# Autodesk Inventor assembly: Head
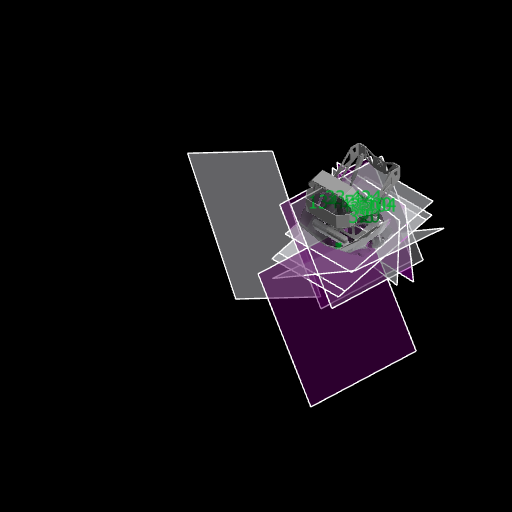
[picture p0: Inventor's stored thumbnail of the model, 512x512]
Saved by Autodesk Inventor 2025.2 (Build 292293000, 293)
## iProperties
Created: 2024-12-17
Part Number: Head
Document SubType Name: Assembly
Designer: valer
Author: valer
## Documents named in this file (47)
- C:\Users\valer\Desktop\str1ker\cad\Head.iam
- C:\Users\valer\Desktop\str1ker\cad\Head.ipt
- C:\Users\valer\Desktop\str1ker\cad\HeadMount.ipt
- C:\Users\valer\Desktop\str1ker\cad\external\DepthSensor\PrimeSenseCarmine1.09.ipt
- C:\Users\valer\Desktop\str1ker\cad\external\HingedThreadedStandoffPart1.ipt
- C:\Users\valer\Desktop\str1ker\cad\external\HingedThreadedStandoffPart2.ipt
- C:\Users\valer\Desktop\str1ker\cad\external\ShaftD6Female-632Female.ipt
- C:\Users\valer\Desktop\str1ker\cad\external\ShaftD6-2101-0006-0160.ipt
- C:\Users\valer\Desktop\str1ker\cad\TongueMount.ipt
- C:\Users\valer\Desktop\str1ker\cad\external\SetScrewLiteHub-1308-0016-0006.ipt
- C:\Users\valer\Desktop\str1ker\cad\external\ShaftD6-Short-2101-0006-0020.ipt
- C:\Users\valer\Desktop\str1ker\cad\external\UJoint6D\UJoint6D-Body-4003-1006-1006.ipt
- C:\Users\valer\Desktop\str1ker\cad\external\UJoint6D\UJoint6D-Screw.ipt
- C:\Users\valer\Desktop\str1ker\cad\external\UJoint6D\UJoint6D-CenterDrive-4003-1006-1006.ipt
- C:\Users\valer\Desktop\str1ker\cad\external\ShaftD6-2100-0006-0200.ipt
- C:\Users\valer\Desktop\str1ker\cad\external\ShaftD6-2101-0006-0140.ipt
- C:\Users\valer\Desktop\str1ker\cad\external\LinearBearing-1612-0612-0035.ipt
- C:\Users\valer\Desktop\str1ker\cad\external\ClampingHub1301-0016-0012.ipt
- C:\Users\valer\Desktop\str1ker\cad\external\ShaftClamp6-6058N14.ipt
- C:\Users\valer\Desktop\str1ker\cad\external\TongueSpeaker.ipt
- C:\Users\valer\Desktop\str1ker\cad\TongueSideLid.ipt
- C:\Users\valer\Desktop\str1ker\cad\TongueSideLidMirror.ipt
- C:\Users\valer\Desktop\str1ker\cad\NoseMount.ipt
- C:\Users\valer\Desktop\str1ker\cad\JawMount.ipt
- C:\Users\valer\Desktop\str1ker\cad\external\93655A703_Male-Female Threaded Hex Standoff.ipt
- C:\Users\valer\Desktop\str1ker\cad\CameraMount.ipt
- C:\Users\valer\Desktop\str1ker\cad\external\ServoHorn-1900-0024-0104.ipt
- C:\Users\valer\Desktop\str1ker\cad\external\ServoCity-2000-0025-0002.ipt
- C:\Users\valer\Desktop\str1ker\cad\external\Beam4-1102-0004-0032.ipt
- C:\Users\valer\Desktop\str1ker\cad\Visor.ipt
- C:\Users\valer\Desktop\str1ker\cad\external\NeckActuator\LA-T8-1215-50 105-64 Body.ipt
- C:\Users\valer\Desktop\str1ker\cad\external\NeckActuator\LA-T8-1215-50 105-64 Shaft.ipt
- C:\Users\valer\Desktop\str1ker\cad\external\NeckActuator\LA-T8-Bracket.ipt
- C:\Users\valer\Desktop\str1ker\cad\NeckBase.ipt
- C:\Users\valer\Desktop\str1ker\cad\NeckBracket.ipt
- C:\Users\valer\Desktop\str1ker\cad\NeckBracketMirror.ipt
- C:\Users\valer\Desktop\str1ker\cad\NeckCover.ipt
- C:\Users\valer\Desktop\str1ker\cad\NeckPotentiometerBracket.ipt
- C:\Users\valer\Desktop\str1ker\cad\external\PololuHub1994.ipt
- C:\Users\valer\Desktop\str1ker\cad\external\rh24pce.iam
- C:\Users\valer\Desktop\str1ker\cad\NeckMiddleBracket.ipt
- C:\Users\valer\Desktop\str1ker\cad\external\Hub8mm.ipt
- C:\Users\valer\Desktop\str1ker\cad\external\am-4180 Lamprey Absolute Encoder Magnet Ring.ipt
- C:\Users\valer\Desktop\str1ker\cad\NeckRingAlign.ipt
- C:\Users\valer\Desktop\str1ker\cad\external\Max9744_20W_ClassD_Amplifier.ipt
- C:\Users\valer\Desktop\str1ker\cad\external\StepperDriver\HiLetgoTB6600HG.ipt
- C:\Users\valer\Desktop\str1ker\cad\external\ArmDriver\IBTMini.ipt
## Components (94 placed, 46 different names)
1. Head:1 — Flush:1, Flush:2, Mate:1, Flush:3, Mate:4, Mate:5, Mate:6, Mate:7, Mate:8, Mate:9, Mate:10, Mate:11, Mate:12, Mate:13, Mate:14, Mate:15, Mate:16, Mate:17, Mate:18, Mate:19, Mate:20, Mate:59, Angle:13, Mate:89, Mate:90, Flush:13, Mate:119, Mate:121, Flush:15, Flush:16, Flush:17, Flush:18, Flush:19, Mate:124, Mate:125, Mate:126, Mate:127, Mate:128, Mate:129, Flush:20, Mate:131, Mate:132, Mate:133, Flush:157, Flush:166, Mate:230
2. HeadMount:1 — Flush:4, Flush:5, Angle:18, Mate:89, Mate:90, Angle:20, Angle:22, Angle:26, Angle:28, Angle:32, Mate:102, Mate:105, Mate:107, Mate:109, Mate:111, Mate:113, Mate:115, Mate:134, Mate:135, Mate:136, Mate:137, Angle:35, Mate:167, Flush:158, Mate:178, Mate:189, Mate:192, Mate:193, Mate:194, Mate:195, Angle:37, Angle:39, Angle:40, Mate:215, Angle:42, Mate:216
3. PrimeSenseCarmine1.09:1 — Flush:6, Flush:23, Mate:138, Mate:198
4. HingedThreadedStandoffPart1:1 — Mate:4, Mate:5, Mate:25, Mate:26
5. HingedThreadedStandoffPart1:2 — Mate:6, Mate:7, Mate:36, Mate:39
6. HingedThreadedStandoffPart1:3 — Mate:8, Mate:9, Mate:37, Mate:38
7. HingedThreadedStandoffPart1:4 — Mate:10, Mate:11, Mate:23, Mate:24
8. HingedThreadedStandoffPart1:5 — Mate:12, Mate:13, Mate:27, Mate:28
9. HingedThreadedStandoffPart1:6 — Mate:16, Mate:17, Mate:29, Mate:40
10. HingedThreadedStandoffPart1:7 — Mate:14, Mate:15, Mate:30, Mate:31
11. HingedThreadedStandoffPart1:8 — Mate:18, Mate:19, Mate:32, Mate:34
12. HingedThreadedStandoffPart1:9 — Mate:20, Mate:33, Mate:35, Mate:59
13. HingedThreadedStandoffPart2:4 — Mate:23, Mate:24, Flush:7, Flush:8
14. HingedThreadedStandoffPart2:5 — Mate:25, Mate:26, Flush:8, Mate:68
15. HingedThreadedStandoffPart2:6 — Mate:27, Mate:28, Flush:7, Flush:10, Mate:69
16. HingedThreadedStandoffPart2:7 — Mate:29, Mate:40, Mate:45, Mate:47
17. HingedThreadedStandoffPart2:8 — Mate:30, Mate:31, Mate:46, Mate:48
18. HingedThreadedStandoffPart2:9 — Mate:32, Mate:34, Mate:49, Mate:52
19. HingedThreadedStandoffPart2:10 — Mate:33, Mate:35, Mate:50, Mate:51
20. HingedThreadedStandoffPart2:11 — Mate:36, Mate:39, Mate:41, Mate:42
21. HingedThreadedStandoffPart2:12 — Mate:37, Mate:38, Mate:43, Mate:44
22. ShaftD6-2100-0006-0200:1 — Mate:87, Angle:17, Mate:88, Angle:18, Mate:108
23. ShaftD6Female-632Female:1 — Mate:41, Mate:42, Mate:87, Angle:17, Mate:88
24. ShaftD6Female-632Female:2 — Mate:43, Mate:44, Mate:91, Mate:92
25. ShaftD6Female-632Female:3 — Mate:45, Mate:47, Mate:95, Mate:96, Angle:23
26. ShaftD6Female-632Female:4 — Mate:46, Mate:48, Mate:93, Mate:94, Angle:21
27. ShaftD6Female-632Female:5 — Mate:49, Mate:52, Mate:99, Mate:100, Angle:30
28. ShaftD6Female-632Female:6 — Mate:50, Mate:51, Mate:97, Mate:98, Angle:27
29. TongueMount:1 — Flush:11, Mate:66, Mate:67, Angle:11, Mate:68, Mate:69, Mate:71
30. SetScrewLiteHub-1308-0016-0006:1 — Mate:66, Mate:67, Angle:11, Mate:70, Mate:73
31. ShaftD6-Short-2101-0006-0020:1 — Mate:70, Mate:71, Mate:72, Angle:12
32. UJoint6D-Body-4003-1006-1006:1 — Mate:72, Mate:73, Angle:12, Mate:74, Mate:75, Mate:76, Mate:77, Mate:78, Mate:79
33. UJoint6D-Screw:1 — Mate:82, Mate:83
34. UJoint6D-CenterDrive-4003-1006-1006:1 — Mate:74, Mate:75, Mate:80, Mate:81
35. UJoint6D-Screw:2 — Mate:76, Mate:77
36. UJoint6D-Screw:3 — Mate:78, Mate:79
37. UJoint6D-Body-4003-1006-1006:2 — Mate:80, Mate:81, Angle:13, Mate:82, Mate:83, Mate:84, Mate:85, Mate:86, Angle:14, Flush:12
38. UJoint6D-Screw:4 — Mate:84, Mate:85
39. ShaftD6-2101-0006-0160:7 — Mate:86, Angle:14, Flush:12, Mate:101, Mate:166, Mate:168
40. ShaftD6-2100-0006-0200:2 — Mate:91, Mate:92, Angle:19, Angle:20, Mate:110
41. ShaftD6-2101-0006-0140:1 — Mate:93, Mate:94, Angle:21, Angle:22, Angle:24, Mate:104
42. ShaftD6-2101-0006-0140:2 — Mate:95, Mate:96, Angle:23, Angle:25, Angle:26, Mate:106
43. ShaftD6-2101-0006-0140:3 — Mate:97, Mate:98, Angle:27, Angle:28, Angle:29, Mate:112
44. ShaftD6-2101-0006-0140:4 — Mate:99, Mate:100, Angle:30, Angle:31, Angle:32, Mate:114
45. LinearBearing-1612-0612-0035:1 — Mate:101, Mate:103, Flush:160
46. ClampingHub1301-0016-0012:1 — Mate:102, Mate:103, Flush:160, Mate:197, Angle:37
47. ShaftClamp6-6058N14:1 — Mate:106, Mate:107
48. ShaftClamp6-6058N14:2 — Mate:104, Mate:105
49. ShaftClamp6-6058N14:3 — Mate:108, Mate:109
50. ShaftClamp6-6058N14:4 — Mate:110, Mate:111
51. ShaftClamp6-6058N14:5 — Mate:114, Mate:115
52. ShaftClamp6-6058N14:6 — Mate:112, Mate:113
53. TongueSpeaker:1 — Mate:119, Mate:122, Mate:123
54. TongueSpeaker:2 — Mate:121, Mate:130
55. TongueSideLid:1 — Mate:124, Mate:125, Mate:126
56. TongueSideLidMirror:1 — Mate:127, Mate:128, Mate:129, Mate:130
57. NoseMount:1 — Flush:21, Mate:131, Mate:132, Mate:133
58. JawMount:1 — Flush:22
59. 93655A703_Male-Female Threaded Hex Standoff:1 — Mate:134, Mate:136, Mate:141, Mate:143
60. 93655A703_Male-Female Threaded Hex Standoff:2 — Mate:135, Mate:137, Mate:142
61. CameraMount:1 — Flush:24, Mate:138, Mate:141, Mate:142, Mate:143, Mate:198
62. ServoHorn-1900-0024-0104:1 — Mate:164, Mate:165, Mate:169, Mate:170
63. ServoCity-2000-0025-0002:1 — Mate:164, Mate:165, Angle:35, Flush:153, Mate:167
64. ShaftClamp6-6058N14:7 — Mate:166, Mate:197
65. ShaftClamp6-6058N14:8 — Mate:168, Mate:171
66. Beam4-1102-0004-0032:1 — Mate:169, Mate:170, Mate:171
67. Visor:1 — Flush:157, Flush:158, Mate:178
68. LA-T8-1215-50 105-64 Body:1 — Mate:172, Mate:175, Mate:179, Mate:180
69. LA-T8-1215-50 105-64 Shaft:1 — Mate:172, Mate:175, Mate:181, Mate:182
70. LA-T8-Bracket:1 — Mate:181, Mate:182, Mate:192, Mate:194, Mate:195, Angle:40
71. LA-T8-Bracket:2 — Mate:179, Mate:180, Mate:206, Mate:237, Angle:47
72. LA-T8-1215-50 105-64 Body:2
73. LA-T8-1215-50 105-64 Shaft:2
74. LA-T8-Bracket:3 — Mate:189, Mate:193, Angle:39
75. LA-T8-Bracket:4 — Mate:238, Angle:46, Mate:249
76. NeckBracket:1 — Mate:206, Mate:237, Mate:239, Mate:240, Mate:241, Mate:244, Angle:47
77. NeckCover:1 — Flush:166
78. NeckCover:2 — Mate:244, Mate:250, Mate:251
79. NeckPotentiometerBracket:1 — Mate:215, Angle:42, Angle:43, Flush:167, Mate:217, Mate:218, Mate:219, Mate:227, Mate:268
80. NeckPotentiometerBracket:2 — Angle:43, Mate:216, Flush:167, Mate:220, Mate:221, Mate:222, Mate:228, Mate:229
81. PololuHub1994:1 — Mate:217, Mate:218, Mate:219
82. PololuHub1994:2 — Mate:220, Mate:221, Mate:222
83. NeckPotentiometerBracket:3 — Mate:227, Flush:168, Mate:268, Mate:269, Mate:270
84. NeckPotentiometerBracket:4 — Mate:228, Mate:229, Flush:168, Mate:266
85. NeckMiddleBracket:1 — Mate:230, Mate:257, Flush:172, Flush:173, Mate:266, Mate:271, Mate:272, Angle:50, Angle:51, Mate:273, Flush:174, Flush:175, Flush:176
86. Hub8mm:1 — Mate:254, Mate:258, Mate:259, Mate:261, Mate:263, Mate:264
87. NeckBase:1 — Mate:238, Mate:239, Mate:240, Mate:241, Mate:246, Mate:247, Mate:248, Mate:254, Mate:255, Mate:258, Mate:259, Mate:262
88. NeckBracketMirror:1 — Mate:246, Mate:247, Mate:248, Angle:46, Mate:249, Mate:250, Mate:251, Mate:257, Flush:172, Flush:173, Mate:275
89. am-4180 Lamprey Absolute Encoder Magnet Ring:1 — Mate:255, Mate:263
90. NeckRingAlign:1 — Mate:261, Mate:262, Mate:264
91. rh24pce:1 [sub-assembly] — Mate:269, Mate:270
92. Max9744_20W_ClassD_Amplifier:1 — Mate:272, Angle:51, Mate:275, Flush:176
93. HiLetgoTB6600HG:1 — Mate:271, Angle:50, Mate:274, Flush:175
94. IBTMini:1 — Mate:273, Mate:274, Flush:174
## Relationships (258: Mate 192, Flush 34, Angle 30, Symmetry 2)
- Flush:1: Head:1
- Flush:2: Head:1
- Mate:1: Head:1
- Flush:3: Head:1
- Flush:4: HeadMount:1
- Flush:5: HeadMount:1
- Flush:6: PrimeSenseCarmine1.09:1
- Mate:4: Head:1 ↔ HingedThreadedStandoffPart1:1
- Mate:5: Head:1 ↔ HingedThreadedStandoffPart1:1
- Mate:6: Head:1 ↔ HingedThreadedStandoffPart1:2
- Mate:7: Head:1 ↔ HingedThreadedStandoffPart1:2
- Mate:8: Head:1 ↔ HingedThreadedStandoffPart1:3
- Mate:9: Head:1 ↔ HingedThreadedStandoffPart1:3
- Mate:10: Head:1 ↔ HingedThreadedStandoffPart1:4
- Mate:11: Head:1 ↔ HingedThreadedStandoffPart1:4
- Mate:12: Head:1 ↔ HingedThreadedStandoffPart1:5
- Mate:13: Head:1 ↔ HingedThreadedStandoffPart1:5
- Mate:14: Head:1 ↔ HingedThreadedStandoffPart1:7
- Mate:15: Head:1 ↔ HingedThreadedStandoffPart1:7
- Mate:16: Head:1 ↔ HingedThreadedStandoffPart1:6
- Mate:17: Head:1 ↔ HingedThreadedStandoffPart1:6
- Mate:18: Head:1 ↔ HingedThreadedStandoffPart1:8
- Mate:19: Head:1 ↔ HingedThreadedStandoffPart1:8
- Mate:20: Head:1 ↔ HingedThreadedStandoffPart1:9
- Mate:23: HingedThreadedStandoffPart1:4 ↔ HingedThreadedStandoffPart2:4
- Mate:24: HingedThreadedStandoffPart1:4 ↔ HingedThreadedStandoffPart2:4
- Mate:25: HingedThreadedStandoffPart1:1 ↔ HingedThreadedStandoffPart2:5
- Mate:26: HingedThreadedStandoffPart1:1 ↔ HingedThreadedStandoffPart2:5
- Mate:27: HingedThreadedStandoffPart1:5 ↔ HingedThreadedStandoffPart2:6
- Mate:28: HingedThreadedStandoffPart1:5 ↔ HingedThreadedStandoffPart2:6
- Mate:29: HingedThreadedStandoffPart1:6 ↔ HingedThreadedStandoffPart2:7
- Mate:30: HingedThreadedStandoffPart1:7 ↔ HingedThreadedStandoffPart2:8
- Mate:31: HingedThreadedStandoffPart1:7 ↔ HingedThreadedStandoffPart2:8
- Mate:32: HingedThreadedStandoffPart1:8 ↔ HingedThreadedStandoffPart2:9
- Mate:33: HingedThreadedStandoffPart1:9 ↔ HingedThreadedStandoffPart2:10
- Mate:34: HingedThreadedStandoffPart1:8 ↔ HingedThreadedStandoffPart2:9
- Mate:35: HingedThreadedStandoffPart1:9 ↔ HingedThreadedStandoffPart2:10
- Mate:36: HingedThreadedStandoffPart1:2 ↔ HingedThreadedStandoffPart2:11
- Mate:37: HingedThreadedStandoffPart1:3 ↔ HingedThreadedStandoffPart2:12
- Mate:38: HingedThreadedStandoffPart1:3 ↔ HingedThreadedStandoffPart2:12
- Mate:39: HingedThreadedStandoffPart1:2 ↔ HingedThreadedStandoffPart2:11
- Mate:40: HingedThreadedStandoffPart1:6 ↔ HingedThreadedStandoffPart2:7
- Flush:7: HingedThreadedStandoffPart2:4 ↔ HingedThreadedStandoffPart2:6
- Flush:8: HingedThreadedStandoffPart2:4 ↔ HingedThreadedStandoffPart2:5
- Mate:41: HingedThreadedStandoffPart2:11 ↔ ShaftD6Female-632Female:1
- Mate:42: HingedThreadedStandoffPart2:11 ↔ ShaftD6Female-632Female:1
- Mate:43: HingedThreadedStandoffPart2:12 ↔ ShaftD6Female-632Female:2
- Mate:44: HingedThreadedStandoffPart2:12 ↔ ShaftD6Female-632Female:2
- Mate:45: HingedThreadedStandoffPart2:7 ↔ ShaftD6Female-632Female:3
- Mate:46: HingedThreadedStandoffPart2:8 ↔ ShaftD6Female-632Female:4
- Mate:47: HingedThreadedStandoffPart2:7 ↔ ShaftD6Female-632Female:3
- Mate:48: HingedThreadedStandoffPart2:8 ↔ ShaftD6Female-632Female:4
- Mate:49: HingedThreadedStandoffPart2:9 ↔ ShaftD6Female-632Female:5
- Mate:50: HingedThreadedStandoffPart2:10 ↔ ShaftD6Female-632Female:6
- Mate:51: HingedThreadedStandoffPart2:10 ↔ ShaftD6Female-632Female:6
- Mate:52: HingedThreadedStandoffPart2:9 ↔ ShaftD6Female-632Female:5
- Mate:59: Head:1 ↔ HingedThreadedStandoffPart1:9
- Flush:10: HingedThreadedStandoffPart2:6
- Flush:11: TongueMount:1
- Mate:66: TongueMount:1 ↔ SetScrewLiteHub-1308-0016-0006:1
- Mate:67: TongueMount:1 ↔ SetScrewLiteHub-1308-0016-0006:1
- Angle:11 (0 deg): TongueMount:1 ↔ SetScrewLiteHub-1308-0016-0006:1
- Mate:68: HingedThreadedStandoffPart2:5 ↔ TongueMount:1
- Mate:69: HingedThreadedStandoffPart2:6 ↔ TongueMount:1
- Mate:70: SetScrewLiteHub-1308-0016-0006:1 ↔ ShaftD6-Short-2101-0006-0020:1
- Mate:71: TongueMount:1 ↔ ShaftD6-Short-2101-0006-0020:1
- Mate:72: ShaftD6-Short-2101-0006-0020:1 ↔ UJoint6D-Body-4003-1006-1006:1
- Mate:73: SetScrewLiteHub-1308-0016-0006:1 ↔ UJoint6D-Body-4003-1006-1006:1
- Angle:12 (0 deg): ShaftD6-Short-2101-0006-0020:1 ↔ UJoint6D-Body-4003-1006-1006:1
- Mate:74: UJoint6D-Body-4003-1006-1006:1 ↔ UJoint6D-CenterDrive-4003-1006-1006:1
- Mate:75: UJoint6D-Body-4003-1006-1006:1 ↔ UJoint6D-CenterDrive-4003-1006-1006:1
- Mate:76: UJoint6D-Body-4003-1006-1006:1 ↔ UJoint6D-Screw:2
- Mate:77: UJoint6D-Body-4003-1006-1006:1 ↔ UJoint6D-Screw:2
- Mate:78: UJoint6D-Body-4003-1006-1006:1 ↔ UJoint6D-Screw:3
- Mate:79: UJoint6D-Body-4003-1006-1006:1 ↔ UJoint6D-Screw:3
- Mate:80: UJoint6D-CenterDrive-4003-1006-1006:1 ↔ UJoint6D-Body-4003-1006-1006:2
- Mate:81: UJoint6D-CenterDrive-4003-1006-1006:1 ↔ UJoint6D-Body-4003-1006-1006:2
- Angle:13 (0 deg): Head:1 ↔ UJoint6D-Body-4003-1006-1006:2
- Mate:82: UJoint6D-Screw:1 ↔ UJoint6D-Body-4003-1006-1006:2
- Mate:83: UJoint6D-Screw:1 ↔ UJoint6D-Body-4003-1006-1006:2
- Mate:84: UJoint6D-Body-4003-1006-1006:2 ↔ UJoint6D-Screw:4
- Mate:85: UJoint6D-Body-4003-1006-1006:2 ↔ UJoint6D-Screw:4
- Mate:86: UJoint6D-Body-4003-1006-1006:2 ↔ ShaftD6-2101-0006-0160:7
- Angle:14 (180 deg): UJoint6D-Body-4003-1006-1006:2 ↔ ShaftD6-2101-0006-0160:7
- Flush:12: UJoint6D-Body-4003-1006-1006:2 ↔ ShaftD6-2101-0006-0160:7
- Mate:87: ShaftD6-2100-0006-0200:1 ↔ ShaftD6Female-632Female:1
- Angle:17 (0 deg): ShaftD6-2100-0006-0200:1 ↔ ShaftD6Female-632Female:1
- Mate:88: ShaftD6-2100-0006-0200:1 ↔ ShaftD6Female-632Female:1
- Angle:18 (0 deg): HeadMount:1 ↔ ShaftD6-2100-0006-0200:1
- Mate:89: Head:1 ↔ HeadMount:1
- Mate:90: Head:1 ↔ HeadMount:1
- Mate:91: ShaftD6Female-632Female:2 ↔ ShaftD6-2100-0006-0200:2
- Mate:92: ShaftD6Female-632Female:2 ↔ ShaftD6-2100-0006-0200:2
- Angle:19 (0 deg): ShaftD6-2100-0006-0200:2
- Angle:20 (0 deg): HeadMount:1 ↔ ShaftD6-2100-0006-0200:2
- Mate:93: ShaftD6Female-632Female:4 ↔ ShaftD6-2101-0006-0140:1
- Mate:94: ShaftD6Female-632Female:4 ↔ ShaftD6-2101-0006-0140:1
- Angle:21 (0 deg): ShaftD6Female-632Female:4 ↔ ShaftD6-2101-0006-0140:1
- Angle:22 (0 deg): HeadMount:1 ↔ ShaftD6-2101-0006-0140:1
- Mate:95: ShaftD6Female-632Female:3 ↔ ShaftD6-2101-0006-0140:2
- Mate:96: ShaftD6Female-632Female:3 ↔ ShaftD6-2101-0006-0140:2
- Angle:23 (0 deg): ShaftD6Female-632Female:3 ↔ ShaftD6-2101-0006-0140:2
- Angle:24 (180 deg): ShaftD6-2101-0006-0140:1
- Angle:25 (180 deg): ShaftD6-2101-0006-0140:2
- Angle:26 (0 deg): HeadMount:1 ↔ ShaftD6-2101-0006-0140:2
- Mate:97: ShaftD6Female-632Female:6 ↔ ShaftD6-2101-0006-0140:3
- Mate:98: ShaftD6Female-632Female:6 ↔ ShaftD6-2101-0006-0140:3
- Angle:27 (0 deg): ShaftD6Female-632Female:6 ↔ ShaftD6-2101-0006-0140:3
- Angle:28 (0 deg): HeadMount:1 ↔ ShaftD6-2101-0006-0140:3
- Angle:29 (0 deg): ShaftD6-2101-0006-0140:3
- Mate:99: ShaftD6Female-632Female:5 ↔ ShaftD6-2101-0006-0140:4
- Mate:100: ShaftD6Female-632Female:5 ↔ ShaftD6-2101-0006-0140:4
- Angle:30 (0 deg): ShaftD6Female-632Female:5 ↔ ShaftD6-2101-0006-0140:4
- Angle:31 (0 deg): ShaftD6-2101-0006-0140:4
- Angle:32 (0 deg): HeadMount:1 ↔ ShaftD6-2101-0006-0140:4
- Mate:101: ShaftD6-2101-0006-0160:7 ↔ LinearBearing-1612-0612-0035:1
- Mate:102: HeadMount:1 ↔ ClampingHub1301-0016-0012:1
- Mate:103: LinearBearing-1612-0612-0035:1 ↔ ClampingHub1301-0016-0012:1
- Mate:104: ShaftD6-2101-0006-0140:1 ↔ ShaftClamp6-6058N14:2
- Mate:105: HeadMount:1 ↔ ShaftClamp6-6058N14:2
- Mate:106: ShaftD6-2101-0006-0140:2 ↔ ShaftClamp6-6058N14:1
- Mate:107: HeadMount:1 ↔ ShaftClamp6-6058N14:1
- Mate:108: ShaftD6-2100-0006-0200:1 ↔ ShaftClamp6-6058N14:3
- Mate:109: HeadMount:1 ↔ ShaftClamp6-6058N14:3
- Mate:110: ShaftD6-2100-0006-0200:2 ↔ ShaftClamp6-6058N14:4
- Mate:111: HeadMount:1 ↔ ShaftClamp6-6058N14:4
- Mate:112: ShaftD6-2101-0006-0140:3 ↔ ShaftClamp6-6058N14:6
- Mate:113: HeadMount:1 ↔ ShaftClamp6-6058N14:6
- Mate:114: ShaftD6-2101-0006-0140:4 ↔ ShaftClamp6-6058N14:5
- Mate:115: HeadMount:1 ↔ ShaftClamp6-6058N14:5
- Flush:13: Head:1
- Mate:119: Head:1 ↔ TongueSpeaker:1
- Mate:121: Head:1 ↔ TongueSpeaker:2
- Flush:15: Head:1
- Flush:16: Head:1
- Symmetry:1
- Mate:122: TongueSpeaker:1
- Flush:17: Head:1
- Flush:18: Head:1
- Symmetry:2
- Mate:123: TongueSpeaker:1
- Flush:19: Head:1
- Mate:124: Head:1 ↔ TongueSideLid:1
- Mate:125: Head:1 ↔ TongueSideLid:1
- Mate:126: Head:1 ↔ TongueSideLid:1
- Mate:127: Head:1 ↔ TongueSideLidMirror:1
- Mate:128: Head:1 ↔ TongueSideLidMirror:1
- Mate:129: Head:1 ↔ TongueSideLidMirror:1
- Mate:130: TongueSpeaker:2 ↔ TongueSideLidMirror:1
- Flush:20: Head:1
- Flush:21: NoseMount:1
- Mate:131: Head:1 ↔ NoseMount:1
- Mate:132: Head:1 ↔ NoseMount:1
- Mate:133: Head:1 ↔ NoseMount:1
- Flush:22: JawMount:1
- Mate:134: HeadMount:1 ↔ 93655A703_Male-Female Threaded Hex Standoff:1
- Mate:135: HeadMount:1 ↔ 93655A703_Male-Female Threaded Hex Standoff:2
- Mate:136: HeadMount:1 ↔ 93655A703_Male-Female Threaded Hex Standoff:1
- Mate:137: HeadMount:1 ↔ 93655A703_Male-Female Threaded Hex Standoff:2
- Flush:23: PrimeSenseCarmine1.09:1
- Flush:24: CameraMount:1
- Mate:138: PrimeSenseCarmine1.09:1 ↔ CameraMount:1
- Mate:141: 93655A703_Male-Female Threaded Hex Standoff:1 ↔ CameraMount:1
- Mate:142: 93655A703_Male-Female Threaded Hex Standoff:2 ↔ CameraMount:1
- Mate:143: 93655A703_Male-Female Threaded Hex Standoff:1 ↔ CameraMount:1
- Mate:164: ServoHorn-1900-0024-0104:1 ↔ ServoCity-2000-0025-0002:1
- Mate:165: ServoHorn-1900-0024-0104:1 ↔ ServoCity-2000-0025-0002:1
- Angle:35 (0 deg): HeadMount:1 ↔ ServoCity-2000-0025-0002:1
- Mate:166: ShaftD6-2101-0006-0160:7 ↔ ShaftClamp6-6058N14:7
- Flush:153: ServoCity-2000-0025-0002:1
- Mate:167 (6 mm): HeadMount:1 ↔ ServoCity-2000-0025-0002:1
- Mate:168: ShaftD6-2101-0006-0160:7 ↔ ShaftClamp6-6058N14:8
- Mate:169: ServoHorn-1900-0024-0104:1 ↔ Beam4-1102-0004-0032:1
- Mate:170: ServoHorn-1900-0024-0104:1 ↔ Beam4-1102-0004-0032:1
- Mate:171: ShaftClamp6-6058N14:8 ↔ Beam4-1102-0004-0032:1
- Flush:157: Head:1 ↔ Visor:1
- Flush:158: HeadMount:1 ↔ Visor:1
- Mate:172: LA-T8-1215-50 105-64 Body:1 ↔ LA-T8-1215-50 105-64 Shaft:1
- Mate:175: LA-T8-1215-50 105-64 Body:1 ↔ LA-T8-1215-50 105-64 Shaft:1
- Mate:178: HeadMount:1 ↔ Visor:1
- Mate:179: LA-T8-1215-50 105-64 Body:1 ↔ LA-T8-Bracket:2
- Mate:180: LA-T8-1215-50 105-64 Body:1 ↔ LA-T8-Bracket:2
- Mate:181: LA-T8-1215-50 105-64 Shaft:1 ↔ LA-T8-Bracket:1
- Mate:182: LA-T8-1215-50 105-64 Shaft:1 ↔ LA-T8-Bracket:1
- [Mate]: LA-T8-1215-50 105-64 Body:2 ↔ LA-T8-1215-50 105-64 Shaft:2
- [Mate]: LA-T8-1215-50 105-64 Body:2 ↔ LA-T8-1215-50 105-64 Shaft:2
- [Mate]: LA-T8-1215-50 105-64 Body:2 ↔ LA-T8-Bracket:4
- [Mate]: LA-T8-1215-50 105-64 Body:2 ↔ LA-T8-Bracket:4
- [Mate]: LA-T8-1215-50 105-64 Shaft:2 ↔ LA-T8-Bracket:3
- [Mate]: LA-T8-1215-50 105-64 Shaft:2 ↔ LA-T8-Bracket:3
- Mate:189: HeadMount:1 ↔ LA-T8-Bracket:3
- Mate:192: HeadMount:1 ↔ LA-T8-Bracket:1
- Mate:193: HeadMount:1 ↔ LA-T8-Bracket:3
- Mate:194: HeadMount:1 ↔ LA-T8-Bracket:1
- Mate:195: HeadMount:1 ↔ LA-T8-Bracket:1
- Flush:160: LinearBearing-1612-0612-0035:1 ↔ ClampingHub1301-0016-0012:1
- Mate:197: ClampingHub1301-0016-0012:1 ↔ ShaftClamp6-6058N14:7
- Mate:198: PrimeSenseCarmine1.09:1 ↔ CameraMount:1
- Angle:37 (0 deg): HeadMount:1 ↔ ClampingHub1301-0016-0012:1
- Angle:39 (0 deg): HeadMount:1 ↔ LA-T8-Bracket:3
- Angle:40 (0 deg): HeadMount:1 ↔ LA-T8-Bracket:1
- Mate:206: LA-T8-Bracket:2 ↔ NeckBracket:1
- Flush:166: Head:1 ↔ NeckCover:1
- Mate:215: HeadMount:1 ↔ NeckPotentiometerBracket:1
- Angle:42 (0 deg): HeadMount:1 ↔ NeckPotentiometerBracket:1
- Angle:43 (0 deg): NeckPotentiometerBracket:1 ↔ NeckPotentiometerBracket:2
- Mate:216: HeadMount:1 ↔ NeckPotentiometerBracket:2
- Flush:167: NeckPotentiometerBracket:1 ↔ NeckPotentiometerBracket:2
- Mate:217: NeckPotentiometerBracket:1 ↔ PololuHub1994:1
- Mate:218: NeckPotentiometerBracket:1 ↔ PololuHub1994:1
- Mate:219: NeckPotentiometerBracket:1 ↔ PololuHub1994:1
- Mate:220: NeckPotentiometerBracket:2 ↔ PololuHub1994:2
- Mate:221: NeckPotentiometerBracket:2 ↔ PololuHub1994:2
- Mate:222: NeckPotentiometerBracket:2 ↔ PololuHub1994:2
- Mate:227: NeckPotentiometerBracket:1 ↔ NeckPotentiometerBracket:3
- Mate:228: NeckPotentiometerBracket:2 ↔ NeckPotentiometerBracket:4
- Mate:229: NeckPotentiometerBracket:2 ↔ NeckPotentiometerBracket:4
- Flush:168: NeckPotentiometerBracket:3 ↔ NeckPotentiometerBracket:4
- Mate:230: Head:1 ↔ NeckMiddleBracket:1
- Mate:237: LA-T8-Bracket:2 ↔ NeckBracket:1
- Mate:238: LA-T8-Bracket:4 ↔ NeckBase:1
- Mate:239: NeckBracket:1 ↔ NeckBase:1
- Mate:240: NeckBracket:1 ↔ NeckBase:1
- Mate:241: NeckBracket:1 ↔ NeckBase:1
- Mate:244: NeckBracket:1 ↔ NeckCover:2
- Mate:246: NeckBase:1 ↔ NeckBracketMirror:1
- Mate:247: NeckBase:1 ↔ NeckBracketMirror:1
- Mate:248: NeckBase:1 ↔ NeckBracketMirror:1
- Angle:46 (0 deg): LA-T8-Bracket:4 ↔ NeckBracketMirror:1
- Angle:47 (0 deg): LA-T8-Bracket:2 ↔ NeckBracket:1
- Mate:249: LA-T8-Bracket:4 ↔ NeckBracketMirror:1
- Mate:250: NeckCover:2 ↔ NeckBracketMirror:1
- Mate:251: NeckCover:2 ↔ NeckBracketMirror:1
- Mate:254: Hub8mm:1 ↔ NeckBase:1
- Mate:255: NeckBase:1 ↔ am-4180 Lamprey Absolute Encoder Magnet Ring:1
- Mate:257: NeckMiddleBracket:1 ↔ NeckBracketMirror:1
- Mate:258: Hub8mm:1 ↔ NeckBase:1
- Mate:259: Hub8mm:1 ↔ NeckBase:1
- Mate:261: Hub8mm:1 ↔ NeckRingAlign:1
- Mate:262: NeckBase:1 ↔ NeckRingAlign:1
- Mate:263: Hub8mm:1 ↔ am-4180 Lamprey Absolute Encoder Magnet Ring:1
- Mate:264: Hub8mm:1 ↔ NeckRingAlign:1
- Flush:172: NeckMiddleBracket:1 ↔ NeckBracketMirror:1
- Flush:173: NeckMiddleBracket:1 ↔ NeckBracketMirror:1
- Mate:266: NeckPotentiometerBracket:4 ↔ NeckMiddleBracket:1
- Mate:268: NeckPotentiometerBracket:1 ↔ NeckPotentiometerBracket:3
- Mate:269: NeckPotentiometerBracket:3 ↔ rh24pce:1
- Mate:270: NeckPotentiometerBracket:3 ↔ rh24pce:1
- Mate:271: NeckMiddleBracket:1 ↔ HiLetgoTB6600HG:1
- Mate:272: NeckMiddleBracket:1 ↔ Max9744_20W_ClassD_Amplifier:1
- Angle:50 (0 deg): NeckMiddleBracket:1 ↔ HiLetgoTB6600HG:1
- Angle:51 (0 deg): NeckMiddleBracket:1 ↔ Max9744_20W_ClassD_Amplifier:1
- Mate:273: NeckMiddleBracket:1 ↔ IBTMini:1
- Mate:274 (15 mm): HiLetgoTB6600HG:1 ↔ IBTMini:1
- Flush:174 (2 mm): NeckMiddleBracket:1 ↔ IBTMini:1
- Flush:175 (2 mm): NeckMiddleBracket:1 ↔ HiLetgoTB6600HG:1
- Mate:275 (10 mm): NeckBracketMirror:1 ↔ Max9744_20W_ClassD_Amplifier:1
- Flush:176 (19 mm): NeckMiddleBracket:1 ↔ Max9744_20W_ClassD_Amplifier:1
## Named parameters: d350_d335 = 0 mm, d351_d342 = 0 mm, d352_d346 = 0 mm, d353_d347 = 0 mm, d354_d348 = 0 mm, d355_d349 = 0 mm
